# Autodesk Inventor assembly: ArmSolenoid
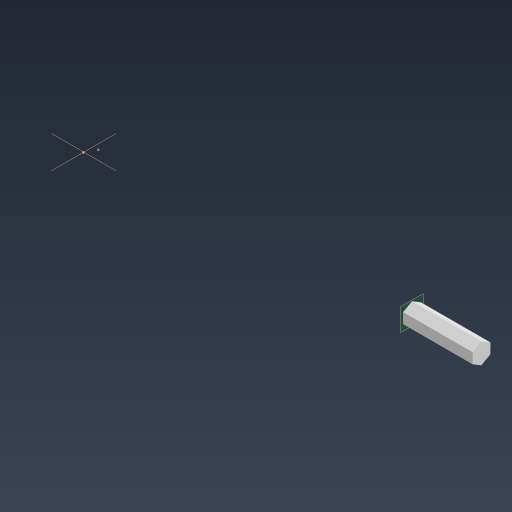
[picture p0: Inventor's stored thumbnail of the model, 512x512]
Saved by Autodesk Inventor 2023 (Build 270158000, 158)
## iProperties
Created: 2023-03-29
Part Number: ArmSolenoid
Document SubType Name: Assembly
Designer: LattePanda
Author: LattePanda
## Documents named in this file (6)
- C:\Users\valer\Desktop\str1ker\cad\ArmSolenoid.iam
- C:\Users\valer\Desktop\str1ker\cad\external\ArmSolenoid\ArmSolenoidBody.ipt
- C:\Users\valer\Desktop\str1ker\cad\SolenoidBracket.ipt
- C:\Users\valer\Desktop\str1ker\cad\external\ArmSolenoid\ArmSolenoidShaft.ipt
- C:\Users\valer\Desktop\str1ker\cad\ArmSolenoidBoundingBox.ipt
- C:\Users\valer\Desktop\str1ker\cad\external\ArmSolenoid\ArmSolenoidShaftBoundingBox.ipt
## Components (5 placed, 5 different names)
1. ArmSolenoid:1 — Mate:11, Mate:12, Mate:13, Mate:14
2. SolenoidBracket:1 — Mate:13, Mate:14, Flush:1, Mate:15, Angle:1, Flush:2, Flush:3, Flush:4, Mate:16
3. ArmSolenoidShaft:1 — Mate:11, Mate:12, Flush:5
4. ArmSolenoidBoundingBox:1 — Flush:2, Flush:3, Flush:4
5. ArmSolenoidShaftBoundingBox:1 — Flush:5, Mate:16, Flush:6
## Relationships (13: Mate 6, Flush 6, Angle 1)
- Mate:11 (6 mm): ArmSolenoid:1 ↔ ArmSolenoidShaft:1
- Mate:12: ArmSolenoid:1 ↔ ArmSolenoidShaft:1
- Mate:13: ArmSolenoid:1 ↔ SolenoidBracket:1
- Mate:14: ArmSolenoid:1 ↔ SolenoidBracket:1
- Flush:1: SolenoidBracket:1
- Mate:15: SolenoidBracket:1
- Angle:1 (0 deg): SolenoidBracket:1
- Flush:2: SolenoidBracket:1 ↔ ArmSolenoidBoundingBox:1
- Flush:3: SolenoidBracket:1 ↔ ArmSolenoidBoundingBox:1
- Flush:4: SolenoidBracket:1 ↔ ArmSolenoidBoundingBox:1
- Flush:5: ArmSolenoidShaft:1 ↔ ArmSolenoidShaftBoundingBox:1
- Mate:16: SolenoidBracket:1 ↔ ArmSolenoidShaftBoundingBox:1
- Flush:6: ArmSolenoidShaftBoundingBox:1
